# Autodesk Inventor assembly: 300-031 (BODY SUPPORT)
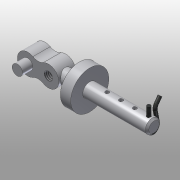
[picture p0: Inventor's stored thumbnail of the model, 180x180]
Saved by Autodesk Inventor 2016 (Build 200138000, 138)
## iProperties
Created: 2015-04-18
Part Number: 300-031 (BODY SUPPORT)
Document SubType Name: Assembly
Designer: Station9
Author: Station9
## Documents named in this file (4)
- E:\worldskills Project\Project Archive\AD\AD-6(94.01.29)WSC2011\300-031 (BODY SUPPORT).iam
- E:\worldskills Project\Project Archive\AD\AD-6(94.01.29)WSC2011\500-178.ipt
- E:\worldskills Project\Project Archive\AD\AD-6(94.01.29)WSC2011\500-177.ipt
- E:\worldskills Project\Project Archive\AD\AD-6(94.01.29)WSC2011\500-179.ipt
## Components (3 placed, 3 different names)
1. 500-178:1 — Mate:1, Mate:2
2. 500-177:1 — Mate:2
3. 500-179:1 — Mate:1
## Relationships (2: Mate 2)
- Mate:1: 500-178:1 ↔ 500-179:1
- Mate:2: 500-178:1 ↔ 500-177:1
